# Autodesk Inventor assembly: Marco_apm_002-4
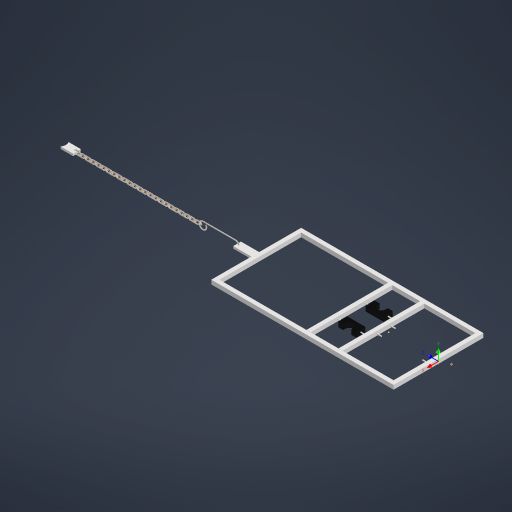
[picture p0: Inventor's stored thumbnail of the model, 512x512]
Saved by Autodesk Inventor 2024 (Build 280153000, 153)
## iProperties
Created: 2023-05-17
Part Number: Marco_apm_002-4
Document SubType Name: Assembly
Designer: javie
Author: javie
## Documents named in this file (9)
- C:\Users\javie\Downloads\Piezas CMR\Marco_APM_002\Marco_apm_002-4.iam
- C:\Users\javie\Downloads\Piezas CMR\Marco_Conveyor_Aereo.iam
- C:\Users\javie\Downloads\Piezas CMR\Marcos_solids\Pieza1.ipt
- C:\Users\javie\Downloads\Piezas CMR\Marcos_solids\Pieza2.ipt
- C:\Users\javie\Downloads\Piezas CMR\Marcos_solids\Topes_apm_002-2.ipt
- C:\Users\javie\Downloads\Piezas CMR\Marcos_solids\S_horizontal.ipt
- C:\Users\javie\Downloads\Piezas CMR\Marco_APM_002\Piezas\APM_002-5.ipt
- C:\Users\javie\Downloads\Piezas CMR\Marcos_solids\Topes_apm_2.ipt
- C:\Users\javie\Downloads\Piezas CMR\Marcos_solids\0110_v2.ipt
## Components (11 placed, 8 different names)
1. Marco_Conveyor_Aereo:1 [sub-assembly] — Nivelación:1, Nivelación:5, Nivelación:6
2. Pieza1:1 — Nivelación:1
3. Pieza2:1
4. Topes_apm_002-2:1 — Insertar:3
5. S_horizontal:1 — Insertar:3, Nivelación:3, Nivelación:4
6. APM_002-5:1 — Insertar:4, Insertar:6
7. APM_002-5:2 — Insertar:5, Insertar:7
8. Topes_apm_2:1 — Nivelación:3, Nivelación:4, Insertar:4, Insertar:5
9. Topes_apm_2:2 — Insertar:6, Insertar:7, Insertar:8
10. S_horizontal:2 — Insertar:8
11. 0110_v2:1 — Nivelación:5, Nivelación:6
## Relationships (11: Insert 6, Flush 5)
- Nivelación:1 [Flush]: Marco_Conveyor_Aereo:1 ↔ Pieza1:1
- Insertar:3: Topes_apm_002-2:1 ↔ S_horizontal:1
- Nivelación:3 [Flush]: S_horizontal:1 ↔ Topes_apm_2:1
- Nivelación:4 [Flush]: S_horizontal:1 ↔ Topes_apm_2:1
- Insertar:4: APM_002-5:1 ↔ Topes_apm_2:1
- Insertar:5: APM_002-5:2 ↔ Topes_apm_2:1
- Insertar:6: APM_002-5:1 ↔ Topes_apm_2:2
- Insertar:7: APM_002-5:2 ↔ Topes_apm_2:2
- Insertar:8: Topes_apm_2:2 ↔ S_horizontal:2
- Nivelación:5 [Flush]: Marco_Conveyor_Aereo:1 ↔ 0110_v2:1
- Nivelación:6 [Flush]: Marco_Conveyor_Aereo:1 ↔ 0110_v2:1
